# Autodesk Inventor assembly: portaherramienta
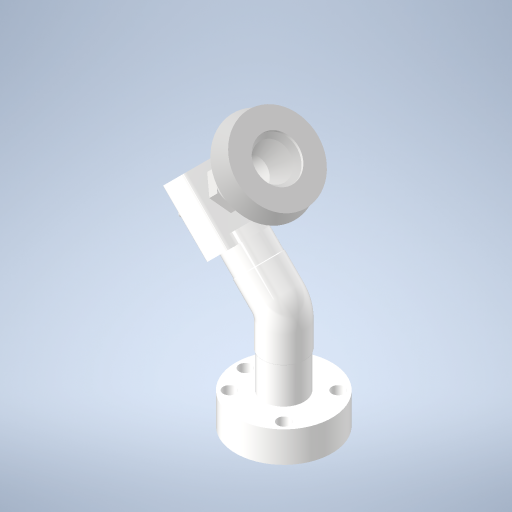
[picture p0: Inventor's stored thumbnail of the model, 512x512]
Saved by Autodesk Inventor 2023 (Build 270158000, 158)
## iProperties
Created: 2022-11-13
Part Number: portaherramienta
Document SubType Name: Assembly
Designer: andre
Author: andre
## Documents named in this file (7)
- C:\Users\andre\Downloads\ProyectoRobotica\CAD\PortaHerramienta\portaherramienta.iam
- C:\Users\andre\Downloads\ProyectoRobotica\CAD\PortaHerramienta\base1.ipt
- C:\Users\andre\Downloads\ProyectoRobotica\CAD\PortaHerramienta\AcopleIntermedio.ipt
- C:\Users\andre\Downloads\ProyectoRobotica\CAD\PortaHerramienta\base2.ipt
- C:\Users\andre\Downloads\ProyectoRobotica\CAD\PortaHerramienta\BaseImpresion.ipt
- C:\Users\andre\Downloads\ProyectoRobotica\CAD\PortaHerramienta\05_02_016.ipt
- C:\Users\andre\Downloads\ProyectoRobotica\CAD\PortaHerramienta\Ventosa.ipt
## Components (6 placed, 6 different names)
1. base1:1 — Rigid:2, Rigid:3, Rigid:5
2. AcopleIntermedio:1 — Rigid:2, Rigid:6
3. base2:1 — Rigid:3
4. BaseImpresion:1 — Rigid:4, Mate:1
5. 05_02_016:1 — Rigid:4, Rigid:5
6. Ventosa:1 — Rigid:6
## Relationships (6: WeldJoint 5, Mate 1)
- Rigid:2 [WeldJoint]: base1:1 ↔ AcopleIntermedio:1
- Rigid:3 [WeldJoint]: base1:1 ↔ base2:1
- Rigid:4 [WeldJoint] (-6.353 mm): BaseImpresion:1 ↔ 05_02_016:1
- Rigid:5 [WeldJoint] (-9 mm): base1:1 ↔ 05_02_016:1
- Rigid:6 [WeldJoint]: AcopleIntermedio:1 ↔ Ventosa:1
- Mate:1: BaseImpresion:1
